# Autodesk Inventor assembly: show case assembly
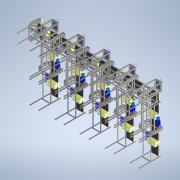
[picture p0: Inventor's stored thumbnail of the model, 180x180]
Saved by Autodesk Inventor 2022.2 (Build 262287010, 287A)
## iProperties
Created: 2022-02-23
Part Number: show case assembly
Document SubType Name: Assembly
Designer: ONG
Author: ONG
## Documents named in this file (6)
- C:\Users\ONG\Documents\INVENTOR DESIGN\音箱\show case assembly.iam
- C:\Users\ONG\Documents\INVENTOR DESIGN\音箱\total asssembly.iam
- C:\Users\ONG\Documents\INVENTOR DESIGN\音箱\conveyour part 2.iam
- C:\Users\ONG\Documents\INVENTOR DESIGN\音箱\conveyour 3.iam
- C:\Users\ONG\Documents\INVENTOR DESIGN\音箱\hydraulic cylinder frame.iam
- C:\Users\ONG\Documents\INVENTOR DESIGN\音箱\total assembly.iam
## Components (21 placed, 5 different names)
1. total assembly:1 [sub-assembly] — Mate:10, Flush:14, Flush:15
2. conveyour part 2:1 [sub-assembly] — Mate:5, Mate:6, Flush:9, Mate:7, Flush:10, Flush:11
3. conveyour part 2:2 [sub-assembly]
4. conveyour part 2:3 [sub-assembly]
5. conveyour part 2:4 [sub-assembly]
6. conveyour part 2:5 [sub-assembly]
7. conveyour 3:1 [sub-assembly] — Mate:7, Flush:10, Flush:11
8. conveyour 3:2 [sub-assembly]
9. conveyour 3:3 [sub-assembly]
10. conveyour 3:4 [sub-assembly]
11. conveyour 3:5 [sub-assembly]
12. hydraulic cylinder frame:1 [sub-assembly] — Flush:13, Mate:8, Mate:9
13. hydraulic cylinder frame:2 [sub-assembly]
14. hydraulic cylinder frame:3 [sub-assembly]
15. hydraulic cylinder frame:4 [sub-assembly]
16. hydraulic cylinder frame:5 [sub-assembly]
17. total asssembly:5 [sub-assembly] — Mate:5, Mate:6, Flush:9, Flush:13, Mate:8, Mate:9, Mate:10, Flush:14, Flush:15
18. total asssembly:6 [sub-assembly]
19. total asssembly:7 [sub-assembly]
20. total asssembly:8 [sub-assembly]
21. total asssembly:9 [sub-assembly]
## Component patterns: (5 elements, first: conveyour part 2:1), (5 elements, first: conveyour 3:1), (5 elements, first: hydraulic cylinder frame:1), (5 elements, first: total asssembly:5)
## Relationships (12: Mate 6, Flush 6)
- Mate:5 (-25 mm): conveyour part 2:1 ↔ total asssembly:5
- Mate:6 (10 mm): conveyour part 2:1 ↔ total asssembly:5
- Flush:9: conveyour part 2:1 ↔ total asssembly:5
- Mate:7 (65 mm): conveyour part 2:1 ↔ conveyour 3:1
- Flush:10: conveyour part 2:1 ↔ conveyour 3:1
- Flush:11: conveyour part 2:1 ↔ conveyour 3:1
- Flush:13: hydraulic cylinder frame:1 ↔ total asssembly:5
- Mate:8 (50 mm): hydraulic cylinder frame:1 ↔ total asssembly:5
- Mate:9 (100 mm): hydraulic cylinder frame:1 ↔ total asssembly:5
- Mate:10: total assembly:1 ↔ total asssembly:5
- Flush:14 (20 mm): total assembly:1 ↔ total asssembly:5
- Flush:15: total assembly:1 ↔ total asssembly:5
